# Autodesk Inventor assembly: batteriesfourpack
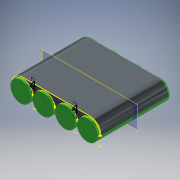
[picture p0: Inventor's stored thumbnail of the model, 180x180]
Saved by Autodesk Inventor 2022.3 (Build 263350000, 350)
## iProperties
Created: 2021-10-06
Part Number: batteriesfourpack
Document SubType Name: Assembly
Designer: Bowen O'Steen
Author: Bowen O'Steen
## Documents named in this file (3)
- C:\Users\gwhen\OneDrive\Documents\Vault\Engineering Data\MemeSat\Subsystems\BoBa\batteriesfourpack.iam
- C:\Users\gwhen\OneDrive\Desktop\Vault\Designs\MEMESat\MemeSat\Engineering Data\MemeSat\Subsystems\BoBa\batterysingle.ipt
- C:\Users\gwhen\OneDrive\Desktop\Vault\Designs\MEMESat\MemeSat\Engineering Data\MemeSat\Subsystems\BoBa\BobaLid.ipt
## Components (5 placed, 2 different names)
1. BobaLid:1 — Mate:3, Mate:4, Mate:5
2. batterysingle:1 — Mate:1, Mate:2, Flush:1, Mate:4, Symmetry:1
3. batterysingle:2
4. batterysingle:3
5. batterysingle:4 — Mate:3, Symmetry:1
## Component patterns: (4 elements, first: batterysingle:1)
## Relationships (7: Mate 5, Flush 1, Symmetry 1)
- Mate:1: batterysingle:1
- Mate:2: batterysingle:1
- Flush:1: batterysingle:1
- Mate:3: BobaLid:1 ↔ batterysingle:4
- Mate:4: BobaLid:1 ↔ batterysingle:1
- Symmetry:1: batterysingle:1 ↔ batterysingle:4
- Mate:5 (-30.425 mm): BobaLid:1
